# Autodesk Inventor assembly: 000 Ensamblaje 3d_LM - Pinza
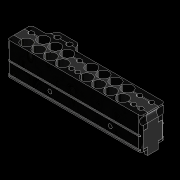
[picture p0: Inventor's stored thumbnail of the model, 180x180]
Saved by Autodesk Inventor 2018.3 (Build 223284000, 284)
## iProperties
Created: 2026-02-10
Part Number: 000 Ensamblaje 3d_LM - Pinza
Document SubType Name: Assembly
Designer: aca6
Author: aca6
## Documents named in this file (5)
- C:\Users\aca6\git\LM\items\hw_LM\variants\items\Welding Tooling\3d\000 Ensamblaje 3d_LM - Pinza.iam
- C:\Users\aca6\git\LM\items\hw_LM\variants\items\Welding Tooling\3d\3d_LM - Pinza 1.ipt
- C:\Users\aca6\git\LM\items\hw_LM\variants\items\Welding Tooling\3d\3d_LM - Pinza 2.ipt
- C:\Users\aca6\git\LM\items\hw_LM\variants\items\Welding Tooling\3d\3d_LM - Pinza 4.ipt
- C:\Users\aca6\git\LM\items\hw_LM\variants\items\Welding Tooling\3d\3d_LM - Pinza 3.ipt
## Components (4 placed, 4 different names)
1. 3d_LM - Pinza 1:1 — Flush:1, Mate:7, Mate:8
2. 3d_LM - Pinza 2:1 — Flush:1, Mate:7, Mate:8, Mate:9, Mate:12, Mate:14
3. 3d_LM - Pinza 4:1 — Mate:10, Mate:11, Mate:13
4. 3d_LM - Pinza 3:1 — Mate:9, Mate:10, Mate:11, Mate:12, Mate:13, Mate:14
## Relationships (9: Mate 8, Flush 1)
- Flush:1: 3d_LM - Pinza 1:1 ↔ 3d_LM - Pinza 2:1
- Mate:7: 3d_LM - Pinza 1:1 ↔ 3d_LM - Pinza 2:1
- Mate:8: 3d_LM - Pinza 1:1 ↔ 3d_LM - Pinza 2:1
- Mate:9: 3d_LM - Pinza 2:1 ↔ 3d_LM - Pinza 3:1
- Mate:10: 3d_LM - Pinza 4:1 ↔ 3d_LM - Pinza 3:1
- Mate:11: 3d_LM - Pinza 4:1 ↔ 3d_LM - Pinza 3:1
- Mate:12: 3d_LM - Pinza 2:1 ↔ 3d_LM - Pinza 3:1
- Mate:13: 3d_LM - Pinza 4:1 ↔ 3d_LM - Pinza 3:1
- Mate:14: 3d_LM - Pinza 2:1 ↔ 3d_LM - Pinza 3:1
